# Autodesk Inventor assembly: Body
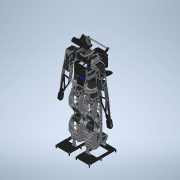
[picture p0: Inventor's stored thumbnail of the model, 180x180]
Saved by Autodesk Inventor 2020 (Build 240168000, 168)
## iProperties
Created: 2021-09-30
Part Number: Body
Document SubType Name: Assembly
Designer: Masato Kubotera
Mass: 4468.65 g
Surface Area: 13553.6 cm^2
Volume: 2294.33 cm^3
Density: 1.94769 g/cm^3
Author: Masato Kubotera
## Documents named in this file (4)
- C:\Users\Masato\Desktop\OpenPlatform_ver3_0\Body.iam
- C:\Users\Masato\Desktop\OpenPlatform_ver3_0\UpperBody\UpperBody.iam
- C:\Users\Masato\Desktop\OpenPlatform_ver3_0\LowerBody\LowerBody.iam
- C:\Users\Masato\Desktop\OpenPlatform_ver3_0\LowerBody\LowerBody_MIR.iam
## Components (3 placed, 3 different names)
1. UpperBody:1 [sub-assembly] — 挿入:1, フラッシュ:1, フラッシュ:2, 挿入:2, 角度:2, 角度:3
2. LowerBody:1 [sub-assembly] — 挿入:1, メイト:1, 角度:2
3. LowerBody_MIR:1 [sub-assembly] — 挿入:2, 角度:3
## Relationships (7: Insert 2, Flush 2, Angle 2, Mate 1)
- 挿入:1 [Insert]: UpperBody:1 ↔ LowerBody:1
- フラッシュ:1 [Flush] (-12 mm): UpperBody:1
- メイト:1 [Mate]: LowerBody:1
- フラッシュ:2 [Flush] (-60 mm): UpperBody:1
- 挿入:2 [Insert]: UpperBody:1 ↔ LowerBody_MIR:1
- 角度:2 [Angle] (0 deg): UpperBody:1 ↔ LowerBody:1
- 角度:3 [Angle] (0 deg): UpperBody:1 ↔ LowerBody_MIR:1
